# Autodesk Inventor assembly: dtandcata
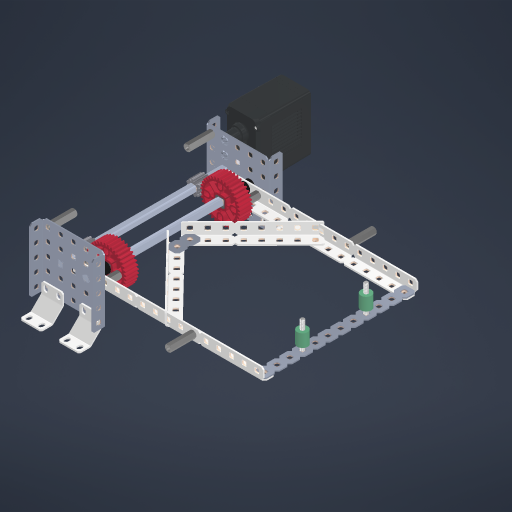
[picture p0: Inventor's stored thumbnail of the model, 512x512]
Saved by Autodesk Inventor 2024 (Build 280153000, 153)
## iProperties
Created: 2023-09-09
Part Number: dtandcata
Document SubType Name: Assembly
Designer: macbook
Author: macbook
## Documents named in this file (24)
- \\Mac\Home\Desktop\code\1599V-VRC\Cad\Assembly\v2\dtandcata.iam
- \\Mac\Home\Desktop\code\1599V-VRC\Cad\Assembly\v2\6wdt.iam
- \\Mac\Home\Desktop\code\1599V-VRC\Cad\Structure\C Channel\old\Steel 1x5x1\Steel C 1x5x1x5.ipt
- \\Mac\Home\Desktop\code\1599V-VRC\Cad\Structure\Gussets\90 Angle Gusset.ipt
- \\Mac\Home\Desktop\code\1599V-VRC\Cad\Motion\Gears\HS Gear\HS 12T Gear, No Insert.iam
- \\Mac\Home\Desktop\code\1599V-VRC\Cad\Motion\Gears\HS Gear.iam
- \\Mac\Home\Desktop\code\1599V-VRC\Cad\Motion\Gears\HS Gear\HS 36T Gear, No Insert.iam
- \\Mac\Home\Desktop\code\1599V-VRC\Cad\Electronics\Motors with Screws\AluM-StarS.iam
- \\Mac\Home\Desktop\code\1599V-VRC\Cad\Electronics\Motors with Screws.iam
- \\Mac\Home\Desktop\code\1599V-VRC\Cad\Structure\Angle\Aluminum\1x1\Alu Angle 1x1x15.ipt
- \\Mac\Home\Desktop\code\1599V-VRC\Cad\Motion\Shaft HS\Shaft HS.ipt
- \\Mac\Home\Desktop\code\1599V-VRC\Cad\Structure\Plate\Steel\Steel Plate 1x12.ipt
- \\Mac\Home\Desktop\code\1599V-VRC\Cad\Field\276-8354-003 Rev2_12-8 Update.ipt
- \\Mac\Home\Desktop\code\1599V-VRC\Cad\Structure\Hardware\Rubber Link.ipt
- \\Mac\Home\Desktop\code\1599V-VRC\Cad\Structure\Plate\Steel\Steel Plate 1x2.ipt
- \\Mac\Home\Desktop\code\1599V-VRC\Cad\Structure\Angle\Aluminum\1x1\Alu Angle 1x1x8.ipt
- \\Mac\Home\Desktop\code\1599V-VRC\Cad\Motion\Shaft HS\HS Spacer\HSpacer .1250.ipt
- \\Mac\Home\Desktop\code\1599V-VRC\Cad\Motion\Shaft HS\HS Spacer.ipt
- \\Mac\Home\Desktop\code\1599V-VRC\Cad\Motion\Shaft HS\HS Spacer\HSpacer .0625.ipt
- \\Mac\Home\Desktop\code\1599V-VRC\Cad\Motion\Shaft HS\HS Spacer\HSpacer .5000.ipt
- \\Mac\Home\Desktop\code\1599V-VRC\Cad\Structure\Standoff\Standoff .50.ipt
- \\Mac\Home\Desktop\code\1599V-VRC\Cad\Structure\Standoff.ipt
- \\Mac\Home\Desktop\code\1599V-VRC\Cad\Structure\Standoff\Standoff 1.00.ipt
- \\Mac\Home\Desktop\code\1599V-VRC\Cad\Motion\Shaft HS\Shaft HS\Shaft HS 6.5 in.ipt
## Components (36 placed, 18 different names)
1. 6wdt:1 [sub-assembly] — Mate:2, Flush:1, Mate:4, Flush:2, Insert:1, Insert:2, Mate:5, Mate:8
2. 90 Angle Gusset:1 — Mate:2, Flush:1
3. 90 Angle Gusset:2 — Mate:4, Flush:2
4. Steel C 1x5x1x5:2 — Insert:1, Rotational:1, Rotational:2, Insert:25, Insert:29, Insert:40
5. Steel C 1x5x1x5:3 — Insert:2, Mate:6, Mate:7, Flush:3, Flush:4, Insert:3, Insert:5, Insert:6, Insert:13, Insert:24, Insert:39
6. 90 Angle Gusset:3 — Mate:5, Mate:6, Flush:3
7. 90 Angle Gusset:4 — Mate:7, Mate:8, Flush:4
8. HS 12T Gear, No Insert:1 [sub-assembly] — Insert:3
9. AluM-StarS:1 [sub-assembly] — Insert:5, Insert:6
10. Alu Angle 1x1x15:1 — Insert:13, Insert:14, Insert:15, Insert:16, Insert:28, Insert:30, Insert:31, Insert:37
11. Shaft HS 6.5 in:1 — Rotational:1, Cylindrical:1
12. Shaft HS 6.5 in:2 — Rotational:2
13. Alu Angle 1x1x15:2 — Insert:11, Insert:12, Insert:17, Cylindrical:1, Insert:27, Insert:32, Insert:33, Insert:38
14. HS 36T Gear, No Insert:4 [sub-assembly] — Insert:11, Insert:12
15. HS 36T Gear, No Insert:5 [sub-assembly] — Insert:14, Insert:15
16. Steel Plate 1x12:2 — Insert:16, Insert:17, Insert:18, Insert:19, Angle:1
17. 276-8354-003 Rev2_12-8 Update:1
18. Rubber Link:1 — Insert:18
19. Rubber Link:2 — Insert:19
20. Alu Angle 1x1x8:2 — Insert:23
21. Alu Angle 1x1x8:1 — Insert:22
22. Steel Plate 1x2:1 — Insert:22, Insert:23, Angle:1
23. HSpacer .1250:1 — Insert:24
24. HSpacer .1250:2 — Insert:25, Insert:26
25. HSpacer .0625:3 — Insert:26
26. HSpacer .5000:4 — Insert:27
27. HSpacer .5000:5 — Insert:28
28. HS 12T Gear, No Insert:6 [sub-assembly] — Insert:29
29. Standoff .50:1 — Insert:30
30. Standoff .50:2 — Insert:31
31. Standoff .50:3 — Insert:33
32. Standoff .50:4 — Insert:32
33. Standoff 1.00:7 — Insert:38
34. Standoff 1.00:8 — Insert:37
35. Standoff 1.00:9 — Insert:39
36. Standoff 1.00:10 — Insert:40
## Relationships (46: Insert 32, Mate 6, Flush 4, RevoluteJoint 2, CylindricalJoint 1, Angle 1)
- Mate:2: 6wdt:1 ↔ 90 Angle Gusset:1
- Flush:1: 6wdt:1 ↔ 90 Angle Gusset:1
- Mate:4: 6wdt:1 ↔ 90 Angle Gusset:2
- Flush:2: 6wdt:1 ↔ 90 Angle Gusset:2
- Insert:1: 6wdt:1 ↔ Steel C 1x5x1x5:2
- Insert:2: 6wdt:1 ↔ Steel C 1x5x1x5:3
- Mate:5: 6wdt:1 ↔ 90 Angle Gusset:3
- Mate:6: Steel C 1x5x1x5:3 ↔ 90 Angle Gusset:3
- Mate:7: Steel C 1x5x1x5:3 ↔ 90 Angle Gusset:4
- Mate:8: 6wdt:1 ↔ 90 Angle Gusset:4
- Flush:3: Steel C 1x5x1x5:3 ↔ 90 Angle Gusset:3
- Flush:4: Steel C 1x5x1x5:3 ↔ 90 Angle Gusset:4
- Insert:3 (19.05 mm): Steel C 1x5x1x5:3 ↔ HS 12T Gear, No Insert:1
- Insert:5: Steel C 1x5x1x5:3 ↔ AluM-StarS:1
- Insert:6: Steel C 1x5x1x5:3 ↔ AluM-StarS:1
- Rotational:1 [RevoluteJoint]: Steel C 1x5x1x5:2 ↔ Shaft HS 6.5 in:1
- Rotational:2 [RevoluteJoint]: Steel C 1x5x1x5:2 ↔ Shaft HS 6.5 in:2
- Insert:11 (12.7 mm): Alu Angle 1x1x15:2 ↔ HS 36T Gear, No Insert:4
- Insert:12 (12.7 mm): Alu Angle 1x1x15:2 ↔ HS 36T Gear, No Insert:4
- Insert:13 (3.175 mm): Steel C 1x5x1x5:3 ↔ Alu Angle 1x1x15:1
- Insert:14 (12.7 mm): Alu Angle 1x1x15:1 ↔ HS 36T Gear, No Insert:5
- Insert:15 (12.7 mm): Alu Angle 1x1x15:1 ↔ HS 36T Gear, No Insert:5
- Insert:16: Alu Angle 1x1x15:1 ↔ Steel Plate 1x12:2
- Insert:17: Alu Angle 1x1x15:2 ↔ Steel Plate 1x12:2
- Cylindrical:1: Shaft HS 6.5 in:1 ↔ Alu Angle 1x1x15:2
- Insert:18 (-4.1275 mm): Steel Plate 1x12:2 ↔ Rubber Link:1
- Insert:19 (-4.1275 mm): Steel Plate 1x12:2 ↔ Rubber Link:2
- [Insert]: Alu Angle 1x1x15:2 ↔ Alu Angle 1x1x8:2
- [Insert]: Alu Angle 1x1x15:1 ↔ Alu Angle 1x1x8:1
- Insert:22: Alu Angle 1x1x8:1 ↔ Steel Plate 1x2:1
- Insert:23: Alu Angle 1x1x8:2 ↔ Steel Plate 1x2:1
- Angle:1 (0 deg): Steel Plate 1x12:2 ↔ Steel Plate 1x2:1
- Insert:24: Steel C 1x5x1x5:3 ↔ HSpacer .1250:1
- Insert:25: Steel C 1x5x1x5:2 ↔ HSpacer .1250:2
- Insert:26: HSpacer .1250:2 ↔ HSpacer .0625:3
- Insert:27: Alu Angle 1x1x15:2 ↔ HSpacer .5000:4
- Insert:28: Alu Angle 1x1x15:1 ↔ HSpacer .5000:5
- Insert:29 (19.05 mm): Steel C 1x5x1x5:2 ↔ HS 12T Gear, No Insert:6
- Insert:30: Alu Angle 1x1x15:1 ↔ Standoff .50:1
- Insert:31: Alu Angle 1x1x15:1 ↔ Standoff .50:2
- Insert:32: Alu Angle 1x1x15:2 ↔ Standoff .50:4
- Insert:33: Alu Angle 1x1x15:2 ↔ Standoff .50:3
- Insert:37: Alu Angle 1x1x15:1 ↔ Standoff 1.00:8
- Insert:38: Alu Angle 1x1x15:2 ↔ Standoff 1.00:7
- Insert:39: Steel C 1x5x1x5:3 ↔ Standoff 1.00:9
- Insert:40: Steel C 1x5x1x5:2 ↔ Standoff 1.00:10
